# Autodesk Inventor assembly: skladacka
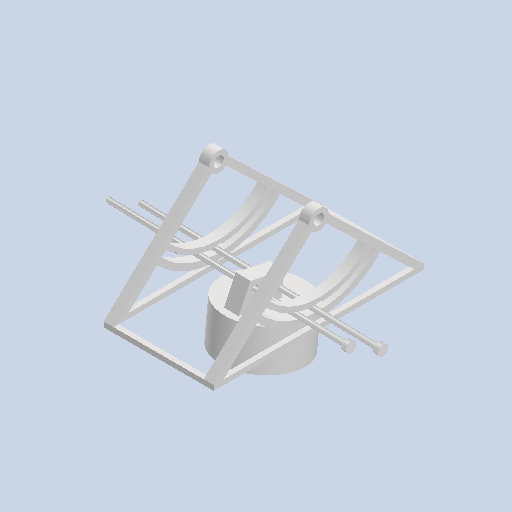
[picture p0: Inventor's stored thumbnail of the model, 512x512]
Saved by Autodesk Inventor 2025 (Build 290162000, 162)
## iProperties
Created: 2025-08-07
Part Number: skladacka
Document SubType Name: Assembly
Designer: Pravoslav
Author: Pravoslav
## Documents named in this file (4)
- D:\Škola\VUT\Igem\šachta\taker\dávkovanie\skladacka.iam
- D:\Škola\VUT\Igem\šachta\taker\dávkovanie\Cage2.ipt
- D:\Škola\VUT\Igem\šachta\taker\dávkovanie\lid2.ipt
- C:\Users\Pravoslav\Documents\Inventor\Content Center Files\R2025\en-US\EP\EP2x100.ipt
## Components (4 placed, 3 different names)
1. Cage2:1
2. lid2:1 — Rigid:1, Mate:1, Mate:2
3. EP 2x100:1 — Rigid:1, Mate:1
4. EP 2x100:2 — Mate:2
## Relationships (3: Mate 2, WeldJoint 1)
- Rigid:1 [WeldJoint]: lid2:1 ↔ EP 2x100:1
- Mate:1: lid2:1 ↔ EP 2x100:1
- Mate:2: lid2:1 ↔ EP 2x100:2
